# Autodesk Inventor assembly: Circular Shooter Assembly
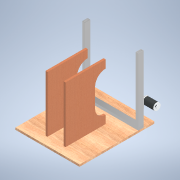
[picture p0: Inventor's stored thumbnail of the model, 180x180]
Saved by Autodesk Inventor 2022.2 (Build 262287000, 287)
## iProperties
Created: 2022-01-19
Part Number: Circular Shooter Assembly
Document SubType Name: Assembly
Designer: robst
Author: robst
## Documents named in this file (7)
- C:\git\CAD-Development\robSteele\2022 Robot\Circular Shooter\Circular Shooter Assembly.iam
- C:\git\CAD-Development\robSteele\2022 Robot\Circular Shooter\basePlate.ipt
- C:\git\CAD-Development\robSteele\2022 Robot\Circular Shooter\baseExtrusion.ipt
- C:\git\CAD-Development\robSteele\2022 Robot\Circular Shooter\sideExtrusion.ipt
- C:\git\CAD-Development\robSteele\2022 Robot\Circular Shooter\am-4244 1IN Bent Bearing Side Mount Gusset.ipt
- C:\git\CAD-Development\robSteele\2022 Robot\Circular Shooter\shooterCircularCurve.ipt
- C:\git\CAD-Development\robSteele\2022 Robot\Circular Shooter\am-0255 2.5inch CIM Motor.ipt
## Components (7 placed, 6 different names)
1. basePlate:1 — Mate:1, Flush:1, Flush:2, Flush:8, Mate:6
2. baseExtrusion:1 — Mate:1, Flush:1, Flush:2, Mate:2, Flush:3, Flush:4, Mate:3, Flush:5, Flush:6, Mate:7
3. sideExtrusion:1 — Mate:2, Flush:3, Flush:4
4. sideExtrusion:2 — Mate:3, Flush:5, Flush:6, Mate:4, Flush:7, Mate:5
5. am-4244 1IN Bent Bearing Side Mount Gusset:1 — Mate:4, Flush:7, Mate:5, Insert:1
6. shooterCircularCurve:1 — Flush:8, Mate:6, Mate:7
7. am-0255 2.5inch CIM Motor:1 — Insert:1
## Relationships (16: Flush 8, Mate 7, Insert 1)
- Mate:1: basePlate:1 ↔ baseExtrusion:1
- Flush:1: basePlate:1 ↔ baseExtrusion:1
- Flush:2 (101.6 mm): basePlate:1 ↔ baseExtrusion:1
- Mate:2: baseExtrusion:1 ↔ sideExtrusion:1
- Flush:3 (76.2 mm): baseExtrusion:1 ↔ sideExtrusion:1
- Flush:4: baseExtrusion:1 ↔ sideExtrusion:1
- Mate:3: baseExtrusion:1 ↔ sideExtrusion:2
- Flush:5: baseExtrusion:1 ↔ sideExtrusion:2
- Flush:6: baseExtrusion:1 ↔ sideExtrusion:2
- Mate:4: sideExtrusion:2 ↔ am-4244 1IN Bent Bearing Side Mount Gusset:1
- Flush:7: sideExtrusion:2 ↔ am-4244 1IN Bent Bearing Side Mount Gusset:1
- Mate:5 (127 mm): sideExtrusion:2 ↔ am-4244 1IN Bent Bearing Side Mount Gusset:1
- Flush:8: basePlate:1 ↔ shooterCircularCurve:1
- Mate:6: basePlate:1 ↔ shooterCircularCurve:1
- Mate:7 (101.6 mm): baseExtrusion:1 ↔ shooterCircularCurve:1
- Insert:1: am-4244 1IN Bent Bearing Side Mount Gusset:1 ↔ am-0255 2.5inch CIM Motor:1
